# Autodesk Inventor assembly: Rotary_system_1
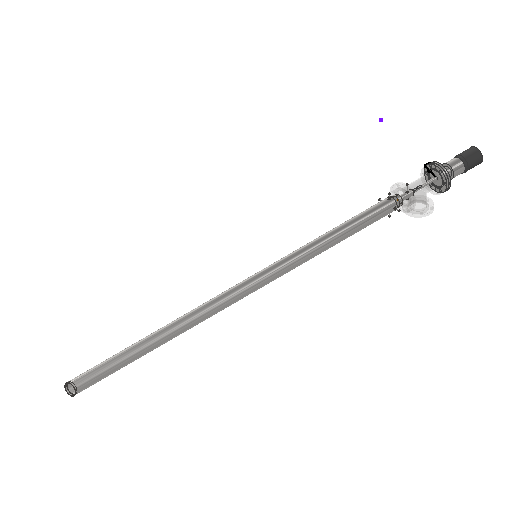
[picture p0: Inventor's stored thumbnail of the model, 512x512]
Saved by Autodesk Inventor 2026.2 (Build 302298000, 298)
## iProperties
Created: 2026-06-01
Part Number: Rotary_system_1
Document SubType Name: Assembly
Designer: zetsu
Author: zetsu
## Documents named in this file (9)
- D:\repos\PIHTI\BoronProbe_5\Figures\Rotary_system_1.iam
- D:\repos\PIHTI\BoronProbe_5\parts\B_probe_pipe_5.ipt
- D:\repos\PIHTI\BoronProbe_5\parts\rotary_transfer_shaft_5_1.ipt
- D:\repos\PIHTI\BoronProbe_5\parts\Rotary_Feedthrough\Rotary_Feedthrough.iam
- D:\repos\PIHTI\BoronProbe_5\parts\M3x10-BHCS.ipt
- D:\repos\PIHTI\BoronProbe_5\parts\M3x20-BHCS.ipt
- D:\repos\PIHTI\BoronProbe_5\parts\M3-nut.ipt
- D:\repos\PIHTI\BoronProbe_5\parts\ceramic_spacer_d3-10.ipt
- D:\repos\PIHTI\BoronProbe_5\parts\ICF70TE\ICF70TE.iam
## Components (14 placed, 7 different names)
1. B_probe_pipe_5:1 — メイト:1, メイト:2, メイト:3, メイト:5, メイト:7, メイト:9, メイト:17, メイト:18, メイト:19, メイト:20
2. rotary_transfer_shaft_5_1:1 — メイト:1, メイト:2, メイト:11, メイト:12, メイト:13, メイト:14, メイト:15, メイト:21, フラッシュ:1, メイト:22, フラッシュ:2, メイト:23, フラッシュ:3, メイト:24, フラッシュ:4
3. Rotary_Feedthrough:1 [sub-assembly] — メイト:11, メイト:12, メイト:25, メイト:26, メイト:27
4. Broached Hexagon Socket Button Head Cap Screw - Metric M3 x 0.5 x 6:1 — メイト:3, メイト:17
5. Broached Hexagon Socket Button Head Cap Screw - Metric M3 x 0.5 x 6:2 — メイト:5, メイト:18
6. Broached Hexagon Socket Button Head Cap Screw - Metric M3 x 0.5 x 6:3 — メイト:7, メイト:20
7. Broached Hexagon Socket Button Head Cap Screw - Metric M3 x 0.5 x 6:4 — メイト:9, メイト:19
8. Broached Hexagon Socket Button Head Cap Screw - Metric M3 x 0.5 x 6:5 — メイト:13, メイト:14, メイト:16
9. JIS B 1181 Style 1 - Metric A M3:1 — メイト:15, メイト:16
10. ceramic_spacer_d3-10:1 — メイト:21, フラッシュ:1
11. ceramic_spacer_d3-10:2 — メイト:22, フラッシュ:2
12. ceramic_spacer_d3-10:3 — メイト:23, フラッシュ:3
13. ceramic_spacer_d3-10:4 — メイト:24, フラッシュ:4
14. ICF70TE:1 [sub-assembly] — メイト:25, メイト:26, メイト:27
## Relationships (27: Mate 23, Flush 4)
- メイト:1 [Mate]: B_probe_pipe_5:1 ↔ rotary_transfer_shaft_5_1:1
- メイト:2 [Mate]: B_probe_pipe_5:1 ↔ rotary_transfer_shaft_5_1:1
- メイト:3 [Mate]: B_probe_pipe_5:1 ↔ Broached Hexagon Socket Button Head Cap Screw - Metric M3 x 0.5 x 6:1
- メイト:5 [Mate]: B_probe_pipe_5:1 ↔ Broached Hexagon Socket Button Head Cap Screw - Metric M3 x 0.5 x 6:2
- メイト:7 [Mate]: B_probe_pipe_5:1 ↔ Broached Hexagon Socket Button Head Cap Screw - Metric M3 x 0.5 x 6:3
- メイト:9 [Mate]: B_probe_pipe_5:1 ↔ Broached Hexagon Socket Button Head Cap Screw - Metric M3 x 0.5 x 6:4
- メイト:11 [Mate]: rotary_transfer_shaft_5_1:1 ↔ Rotary_Feedthrough:1
- メイト:12 [Mate]: rotary_transfer_shaft_5_1:1 ↔ Rotary_Feedthrough:1
- メイト:13 [Mate]: rotary_transfer_shaft_5_1:1 ↔ Broached Hexagon Socket Button Head Cap Screw - Metric M3 x 0.5 x 6:5
- メイト:14 [Mate]: rotary_transfer_shaft_5_1:1 ↔ Broached Hexagon Socket Button Head Cap Screw - Metric M3 x 0.5 x 6:5
- メイト:15 [Mate]: rotary_transfer_shaft_5_1:1 ↔ JIS B 1181 Style 1 - Metric A M3:1
- メイト:16 [Mate]: Broached Hexagon Socket Button Head Cap Screw - Metric M3 x 0.5 x 6:5 ↔ JIS B 1181 Style 1 - Metric A M3:1
- メイト:17 [Mate]: B_probe_pipe_5:1 ↔ Broached Hexagon Socket Button Head Cap Screw - Metric M3 x 0.5 x 6:1
- メイト:18 [Mate]: B_probe_pipe_5:1 ↔ Broached Hexagon Socket Button Head Cap Screw - Metric M3 x 0.5 x 6:2
- メイト:19 [Mate]: B_probe_pipe_5:1 ↔ Broached Hexagon Socket Button Head Cap Screw - Metric M3 x 0.5 x 6:4
- メイト:20 [Mate]: B_probe_pipe_5:1 ↔ Broached Hexagon Socket Button Head Cap Screw - Metric M3 x 0.5 x 6:3
- メイト:21 [Mate]: rotary_transfer_shaft_5_1:1 ↔ ceramic_spacer_d3-10:1
- フラッシュ:1 [Flush]: rotary_transfer_shaft_5_1:1 ↔ ceramic_spacer_d3-10:1
- メイト:22 [Mate]: rotary_transfer_shaft_5_1:1 ↔ ceramic_spacer_d3-10:2
- フラッシュ:2 [Flush]: rotary_transfer_shaft_5_1:1 ↔ ceramic_spacer_d3-10:2
- メイト:23 [Mate]: rotary_transfer_shaft_5_1:1 ↔ ceramic_spacer_d3-10:3
- フラッシュ:3 [Flush]: rotary_transfer_shaft_5_1:1 ↔ ceramic_spacer_d3-10:3
- メイト:24 [Mate]: rotary_transfer_shaft_5_1:1 ↔ ceramic_spacer_d3-10:4
- フラッシュ:4 [Flush]: rotary_transfer_shaft_5_1:1 ↔ ceramic_spacer_d3-10:4
- メイト:25 [Mate]: Rotary_Feedthrough:1 ↔ ICF70TE:1
- メイト:26 [Mate]: Rotary_Feedthrough:1 ↔ ICF70TE:1
- メイト:27 [Mate]: Rotary_Feedthrough:1 ↔ ICF70TE:1
